# Autodesk Inventor assembly: Housing
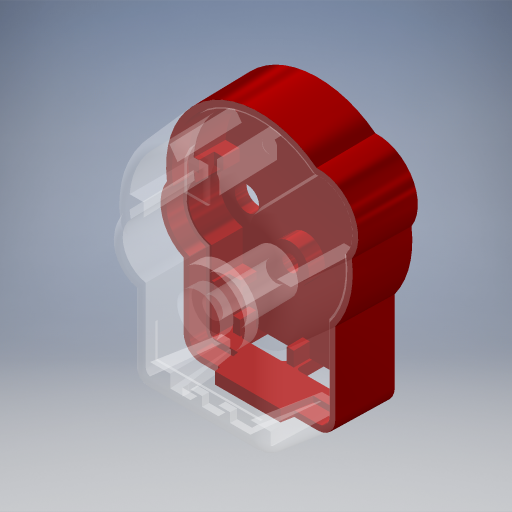
[picture p0: Inventor's stored thumbnail of the model, 512x512]
Saved by Autodesk Inventor 2024.2 (Build 282272000, 272)
## iProperties
Created: 2019-11-27
Part Number: Housing
Description: STEP AP214
Document SubType Name: Assembly
Designer: rohan
Sending System: SolidWorks 2015
Preprocessor: SwSTEP 2.0
Title: Housing.STEP
Revision Number: ANY
## Documents named in this file (3)
- C:\Users\rohan\OneDrive - Hillsborough County Public Schools\Robotics\FIRST-Robotics-Competition\Crescendo\Minotaur-Crescendo-Robot\Structure\3D-Printed-Components\CANcoder-Housing.iam
- C:\Users\rohan\OneDrive - Hillsborough County Public Schools\Robotics\FIRST-Robotics-Competition\Crescendo\Minotaur-Crescendo-Robot\Structure\3D-Printed-Components\CANcoder-Housing\top_rev_E.ipt
- C:\Users\rohan\OneDrive - Hillsborough County Public Schools\Robotics\FIRST-Robotics-Competition\Crescendo\Minotaur-Crescendo-Robot\Structure\3D-Printed-Components\CANcoder-Housing\cover rev_D.ipt
## Components (2 placed, 2 different names)
1. top_rev_E_1 — Mate:1, Mate:2
2. cover rev_D_2 — Mate:1, Mate:2
## Relationships (2: Mate 2)
- Mate:1: top_rev_E_1 ↔ cover rev_D_2
- Mate:2: top_rev_E_1 ↔ cover rev_D_2
